# Autodesk Inventor assembly: CL7-100
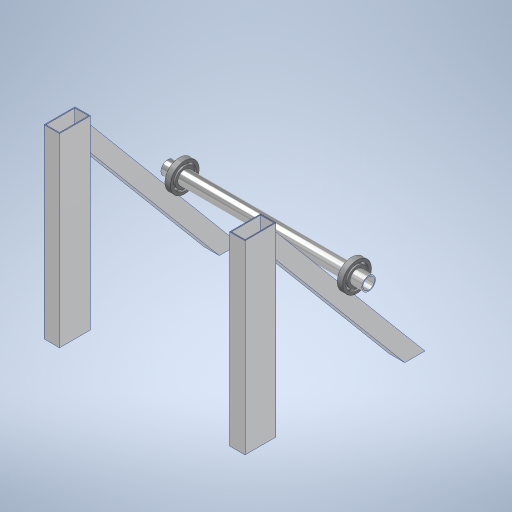
[picture p0: Inventor's stored thumbnail of the model, 512x512]
Saved by Autodesk Inventor 2023.4 (Build 274418000, 418)
## iProperties
Created: 2025-03-17
Part Number: CL7-100
Document SubType Name: Assembly
Designer: dlangdon
Author: dlangdon
## Documents named in this file (5)
- C:\Users\dlangdon\Documents\GitHub\2025-ReefScape---CAD\Climber\CL7\CL7-100.iam
- C:\Users\dlangdon\Documents\GitHub\2025-ReefScape---CAD\Climber\CL7\CL7-001.ipt
- C:\Users\dlangdon\Documents\GitHub\2025-ReefScape---CAD\Climber\CL7\CL-002.ipt
- C:\Users\dlangdon\Documents\GitHub\2025-ReefScape---CAD\Climber\CL7\CL7-003.ipt
- C:\Users\dlangdon\Documents\GitHub\2025-ReefScape---CAD\COMMON PARTS\BEARINGS\0_875_ID_1_875OD_0_375_Thick60355K508_Ball Bearing.ipt
## Components (7 placed, 4 different names)
1. CL7-001:1 — Flush:1, Flush:2, Mate:1, Mate:2, Flush:3, Flush:4
2. CL7-001:2 — Flush:1, Flush:2, Mate:1, Mate:3, Flush:5, Flush:6
3. CL-002:1 — Mate:2, Flush:3, Flush:4
4. CL-002:2 — Mate:3, Flush:5, Flush:6
5. CL7-003:1 — Mate:4, Mate:5
6. 0_875_ID_1_875OD_0_375_Thick60355K508_Ball Bearing:1 — Mate:4, Symmetry:1
7. 0_875_ID_1_875OD_0_375_Thick60355K508_Ball Bearing:2 — Mate:5, Symmetry:1
## Relationships (12: Flush 6, Mate 5, Symmetry 1)
- Flush:1: CL7-001:1 ↔ CL7-001:2
- Flush:2: CL7-001:1 ↔ CL7-001:2
- Mate:1 (279.4 mm): CL7-001:1 ↔ CL7-001:2
- Mate:2: CL7-001:1 ↔ CL-002:1
- Flush:3: CL7-001:1 ↔ CL-002:1
- Flush:4: CL7-001:1 ↔ CL-002:1
- Mate:3: CL7-001:2 ↔ CL-002:2
- Flush:5: CL7-001:2 ↔ CL-002:2
- Flush:6: CL7-001:2 ↔ CL-002:2
- Mate:4: CL7-003:1 ↔ 0_875_ID_1_875OD_0_375_Thick60355K508_Ball Bearing:1
- Mate:5: CL7-003:1 ↔ 0_875_ID_1_875OD_0_375_Thick60355K508_Ball Bearing:2
- Symmetry:1: 0_875_ID_1_875OD_0_375_Thick60355K508_Ball Bearing:1 ↔ 0_875_ID_1_875OD_0_375_Thick60355K508_Ball Bearing:2
